# Autodesk Inventor assembly: Assembly_XYZ_Stage_Micrometer_ontop_lightsheet
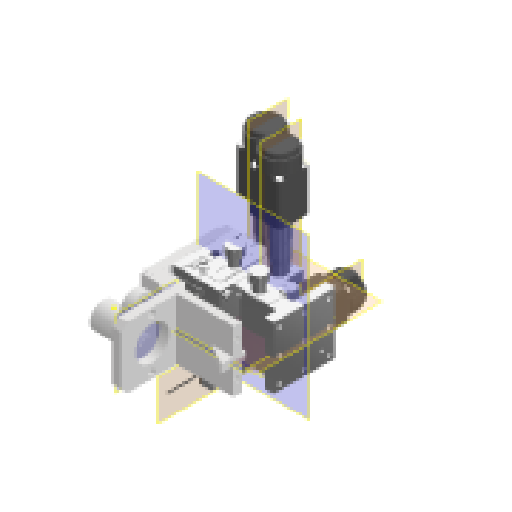
[picture p0: Inventor's stored thumbnail of the model, 512x512]
Saved by Autodesk Inventor 2024.1 (Build 281209000, 209)
## iProperties
Created: 2023-02-07
Part Number: Assembly_XYZ_Stage_Micrometer_ontop_lightsheet
Document SubType Name: Assembly
Designer: diederichbenedict
Author: diederichbenedict
## Documents named in this file (6)
- C:\Users\diederichbenedict\Dropbox\Dokumente\Promotion\PROJECTS\openUC2_SOOP\INVENTOR\Workspace\Assembly_XYZ_Stage_Micrometer_ontop_lightsheet.iam
- C:\Users\diederichbenedict\Dropbox\Dokumente\Promotion\PROJECTS\openUC2_SOOP\INVENTOR\Workspace\00_XYZstage_micro_LT-4047-S1.ipt
- C:\Users\diederichbenedict\Dropbox\Dokumente\Promotion\PROJECTS\openUC2_SOOP\INVENTOR\Workspace\00_Joy-IT-B20SHD4353_NEMA8_captive.ipt
- C:\Users\diederichbenedict\Dropbox\Dokumente\Promotion\PROJECTS\openUC2_SOOP\INVENTOR\Workspace\40_XYZstage_micrometer_motorized_nema8_lightsheet_samplemount_ontop.ipt
- C:\Users\diederichbenedict\Dropbox\Dokumente\Promotion\PROJECTS\openUC2_SOOP\INVENTOR\Workspace\20_Cube_Insert_Lightsheet_syringe_Rotating_hollomotor_nut_v0.ipt
- C:\Users\diederichbenedict\Dropbox\Dokumente\Promotion\PROJECTS\openUC2_SOOP\INVENTOR\Workspace\40_XYZstage_micrometer_motorized_nema8_samplemount_lightsheet_screwed.ipt
## Components (7 placed, 5 different names)
1. 00_XYZstage_micro_LT-4047-S1:1 — Fluchtend:3, Fluchtend:4, Einfügen:6, Winkel:1
2. 00_Joy-IT-B20SHD4353_NEMA8_captive:2
3. 00_Joy-IT-B20SHD4353_NEMA8_captive:1
4. 00_Joy-IT-B20SHD4353_NEMA8_captive:3
5. 40_XYZstage_micrometer_motorized_nema8_lightsheet_samplemount_ontop:1 — Fluchtend:3, Fluchtend:4
6. 20_Cube_Insert_Lightsheet_syringe_Rotating_hollomotor_nut_v0:1
7. 40_XYZstage_micrometer_motorized_nema8_samplemount_lightsheet_screwed:1 — Einfügen:6, Winkel:1
## Relationships (7: Insert 4, Flush 2, Angle 1)
- [Insert]: 00_XYZstage_micro_LT-4047-S1:1 ↔ 00_Joy-IT-B20SHD4353_NEMA8_captive:1
- [Insert]: 00_XYZstage_micro_LT-4047-S1:1 ↔ 00_Joy-IT-B20SHD4353_NEMA8_captive:2
- [Insert]: 00_XYZstage_micro_LT-4047-S1:1 ↔ 00_Joy-IT-B20SHD4353_NEMA8_captive:3
- Fluchtend:3 [Flush]: 00_XYZstage_micro_LT-4047-S1:1 ↔ 40_XYZstage_micrometer_motorized_nema8_lightsheet_samplemount_ontop:1
- Fluchtend:4 [Flush]: 00_XYZstage_micro_LT-4047-S1:1 ↔ 40_XYZstage_micrometer_motorized_nema8_lightsheet_samplemount_ontop:1
- Einfügen:6 [Insert]: 00_XYZstage_micro_LT-4047-S1:1 ↔ 40_XYZstage_micrometer_motorized_nema8_samplemount_lightsheet_screwed:1
- Winkel:1 [Angle] (180 deg): 00_XYZstage_micro_LT-4047-S1:1 ↔ 40_XYZstage_micrometer_motorized_nema8_samplemount_lightsheet_screwed:1
